# Autodesk Inventor assembly: Base2
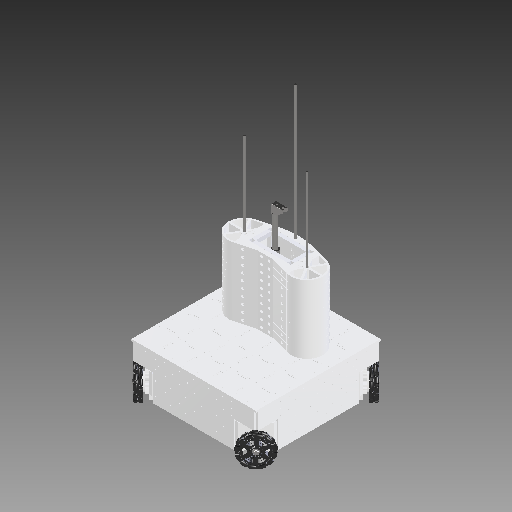
[picture p0: Inventor's stored thumbnail of the model, 512x512]
Saved by Autodesk Inventor 2017 SP1 (Build 210196100, 196)
## iProperties
Created: 2017-06-13
Part Number: Base2
Document SubType Name: Assembly
Designer: zallen
Author: zallen
## Documents named in this file (13)
- C:\Users\Zach\Documents\GitHub\cr-laundry-robot\src\Base\Base.iam
- C:\Users\Zach\Documents\GitHub\cr-laundry-robot\src\Base\Chassis\Chassis.iam
- C:\Users\Zach\Documents\GitHub\cr-laundry-robot\lib\Linear Actuator 300mm\LinearActuator300mm.iam
- C:\Users\Zach\Documents\GitHub\cr-laundry-robot\src\Base\Wheel Assembly\Wheel Assembly.iam
- C:\Users\Zach\Documents\GitHub\cr-laundry-robot\src\Base\Quick Shaft 10mm x 750mm.ipt
- C:\Users\Zach\Documents\GitHub\cr-laundry-robot\lib\ExpertPower EXP12180 Battery.ipt
- C:\Users\Zach\Documents\GitHub\cr-laundry-robot\src\Base\Battery Box\BatteryBox.iam
- C:\Users\Zach\Documents\GitHub\cr-laundry-robot\src\Base\Side Panel\Side Panel.iam
- C:\Users\Zach\Documents\GitHub\cr-laundry-robot\src\Base\Side Panel\Side Panel Front.iam
- C:\Users\Zach\Documents\GitHub\cr-laundry-robot\src\Base\Side Panel\Side Panel Back.iam
- C:\Users\Zach\Documents\GitHub\cr-laundry-robot\src\Base\Rise Base Assembly\Riser Base.iam
- C:\Users\Zach\Documents\GitHub\cr-laundry-robot\src\Base\Top Cover Assembly\Top Cover Assembly.iam
- C:\Users\Zach\Documents\GitHub\cr-laundry-robot\src\Base\Quick Shaft 10mm x 1000mm.ipt
## Components (17 placed, 12 different names)
1. Chassis:1 [sub-assembly] — Mate:36, Mate:37, Mate:38, Mate:39, Mate:40, Mate:41, Mate:42, Mate:43, Mate:44, Mate:45, Mate:46, Mate:47, Mate:48, Mate:49, Mate:165, Flush:63, Mate:166, Flush:64, Mate:168, Mate:169, Mate:174, Mate:175, Mate:176, Mate:177, Mate:178, Mate:179, Mate:181, Mate:184, Mate:185, Mate:197, Mate:198, Mate:199
2. LinearActuator300mm:1 [sub-assembly] — Mate:197, Mate:198, Mate:199
3. Wheel Assembly:1 [sub-assembly] — Mate:36, Mate:37, Mate:38, Mate:39, Mate:40
4. Wheel Assembly:2 [sub-assembly] — Mate:41, Mate:42, Mate:43
5. Wheel Assembly:3 [sub-assembly] — Mate:44, Mate:45, Mate:46
6. Wheel Assembly:4 [sub-assembly] — Mate:47, Mate:48, Mate:49
7. Quick Shaft 10mm x 750mm:1 — Flush:62, Mate:172, Mate:187
8. Quick Shaft 10mm x 750mm:2 — Flush:62, Mate:173, Mate:186, Mate:221
9. Quick Shaft 10mm x 1000mm:1 — Mate:219, Mate:220
10. ExpertPower EXP12180 Battery:1 — Mate:165, Mate:167, Mate:168
11. BatteryBox:1 [sub-assembly] — Flush:63, Mate:166, Flush:64, Mate:167
12. Side Panel:3 [sub-assembly] — Mate:174, Mate:175, Mate:193
13. Side Panel:4 [sub-assembly] — Mate:178, Mate:179, Mate:180
14. Side Panel Front:1 [sub-assembly] — Mate:176, Mate:177
15. Side Panel Back:1 [sub-assembly] — Mate:180, Mate:181, Mate:194
16. Riser Base:1 [sub-assembly] — Mate:184, Mate:185, Mate:186, Mate:187, Mate:219
17. Top Cover Assembly:1 [sub-assembly] — Mate:193, Mate:194, Mate:220, Mate:221
## Relationships (44: Mate 41, Flush 3)
- Mate:36: Chassis:1 ↔ Wheel Assembly:1
- Mate:37: Chassis:1 ↔ Wheel Assembly:1
- Mate:38: Chassis:1 ↔ Wheel Assembly:1
- Mate:39: Chassis:1 ↔ Wheel Assembly:1
- Mate:40: Chassis:1 ↔ Wheel Assembly:1
- Mate:41: Chassis:1 ↔ Wheel Assembly:2
- Mate:42: Chassis:1 ↔ Wheel Assembly:2
- Mate:43: Chassis:1 ↔ Wheel Assembly:2
- Mate:44: Chassis:1 ↔ Wheel Assembly:3
- Mate:45: Chassis:1 ↔ Wheel Assembly:3
- Mate:46: Chassis:1 ↔ Wheel Assembly:3
- Mate:47: Chassis:1 ↔ Wheel Assembly:4
- Mate:48: Chassis:1 ↔ Wheel Assembly:4
- Mate:49: Chassis:1 ↔ Wheel Assembly:4
- Flush:62: Quick Shaft 10mm x 750mm:1 ↔ Quick Shaft 10mm x 750mm:2
- Mate:165: Chassis:1 ↔ ExpertPower EXP12180 Battery:1
- Flush:63: Chassis:1 ↔ BatteryBox:1
- Mate:166: Chassis:1 ↔ BatteryBox:1
- Flush:64: Chassis:1 ↔ BatteryBox:1
- Mate:167: ExpertPower EXP12180 Battery:1 ↔ BatteryBox:1
- Mate:168: Chassis:1 ↔ ExpertPower EXP12180 Battery:1
- Mate:169: Chassis:1
- Mate:172: Quick Shaft 10mm x 750mm:1
- Mate:173: Quick Shaft 10mm x 750mm:2
- Mate:174: Chassis:1 ↔ Side Panel:3
- Mate:175: Chassis:1 ↔ Side Panel:3
- Mate:176: Chassis:1 ↔ Side Panel Front:1
- Mate:177: Chassis:1 ↔ Side Panel Front:1
- Mate:178: Chassis:1 ↔ Side Panel:4
- Mate:179: Chassis:1 ↔ Side Panel:4
- Mate:180: Side Panel:4 ↔ Side Panel Back:1
- Mate:181: Chassis:1 ↔ Side Panel Back:1
- Mate:184: Chassis:1 ↔ Riser Base:1
- Mate:185: Chassis:1 ↔ Riser Base:1
- Mate:186: Quick Shaft 10mm x 750mm:2 ↔ Riser Base:1
- Mate:187: Quick Shaft 10mm x 750mm:1 ↔ Riser Base:1
- Mate:193: Side Panel:3 ↔ Top Cover Assembly:1
- Mate:194: Side Panel Back:1 ↔ Top Cover Assembly:1
- Mate:197: Chassis:1 ↔ LinearActuator300mm:1
- Mate:198: Chassis:1 ↔ LinearActuator300mm:1
- Mate:199: Chassis:1 ↔ LinearActuator300mm:1
- Mate:219: Quick Shaft 10mm x 1000mm:1 ↔ Riser Base:1
- Mate:220: Quick Shaft 10mm x 1000mm:1 ↔ Top Cover Assembly:1
- Mate:221: Quick Shaft 10mm x 750mm:2 ↔ Top Cover Assembly:1
